# Autodesk Inventor assembly: ElevShortBackFrame
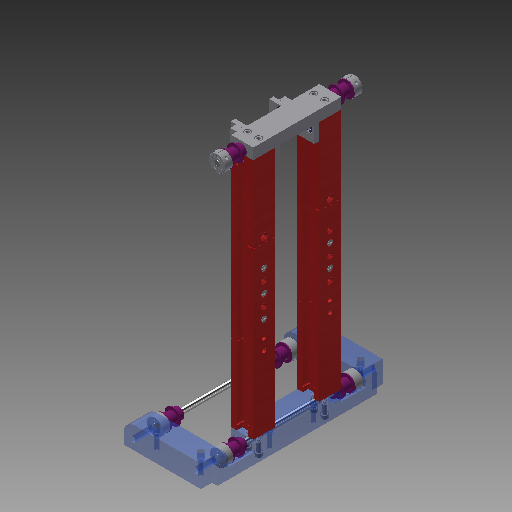
[picture p0: Inventor's stored thumbnail of the model, 512x512]
Saved by Autodesk Inventor 2019 (Build 230136000, 136)
## iProperties
Created: 2019-09-29
Part Number: ElevShortBackFrame
Document SubType Name: Weldment
Designer: james
Weld Material: Welded Aluminum-6061
Author: james
## Documents named in this file (9)
- F:\JimsDesign\Jims2020FTC\ElevShortBackFrame.iam
- F:\JimsDesign\Jims2020FTC\FullElevatorShart.iam
- F:\JimsDesign\Jims2020FTC\ElevBase.ipt
- F:\JimsDesign\Library\McMaster\SocketScrews\91251A201_BLACK-OXIDE ALLOY STEEL SOCKET HEAD SCREW.ipt
- F:\JimsDesign\Jims2020FTC\ElvatorEnd.iam
- F:\JimsDesign\Library\McMaster\Screws\91771A196_18-8 SS FLAT HEAD PHILLIPS MACHINE SCREW.ipt
- F:\JimsDesign\Jims2020FTC\SliderLeft.iam
- F:\JimsDesign\Jims2020FTC\SliderRight.iam
- F:\JimsDesign\Jims2020FTC\EvelShortBackBeam.iam
## Components (17 placed, 8 different names)
1. FullElevatorShart:1 [sub-assembly] — Mate:30, Mate:31
2. ElevBase:1 — Mate:11, Mate:12, Mate:13, Mate:14, Mate:15, Mate:16, Mate:17, Mate:18, Mate:19, Mate:20, Mate:26, Mate:33
3. FullElevatorShart:2 [sub-assembly] — Mate:11, Mate:12
4. EvelShortBackBeam:1 [sub-assembly] — Mate:22, Mate:25, Mate:26, Mate:28, Mate:29, Mate:38, Mate:39, Flush:1, Flush:2, Mate:44, Mate:45, Mate:46
5. EvelShortBackBeam:2 [sub-assembly] — Mate:34, Mate:35, Mate:36, Mate:37, Mate:40, Flush:3, Flush:4, Mate:41, Mate:42, Mate:43
6. 91251A201_BLACK-OXIDE ALLOY STEEL SOCKET HEAD SCREW:1 — Mate:16, Mate:17
7. 91251A201_BLACK-OXIDE ALLOY STEEL SOCKET HEAD SCREW:2 — Mate:15, Mate:19, Mate:22
8. 91251A201_BLACK-OXIDE ALLOY STEEL SOCKET HEAD SCREW:3 — Mate:14, Mate:20, Mate:25
9. 91251A201_BLACK-OXIDE ALLOY STEEL SOCKET HEAD SCREW:4 — Mate:13, Mate:18
10. ElvatorEnd:1 [sub-assembly] — Mate:28, Mate:29, Mate:30, Mate:31, Mate:32, Mate:34, Mate:35, Mate:36
11. FullElevatorShart:3 [sub-assembly] — Mate:32, Mate:33
12. 91771A196_18-8 SS FLAT HEAD PHILLIPS MACHINE SCREW:1 — Mate:39, Flush:2
13. 91771A196_18-8 SS FLAT HEAD PHILLIPS MACHINE SCREW:2 — Mate:38, Flush:1
14. 91771A196_18-8 SS FLAT HEAD PHILLIPS MACHINE SCREW:3 — Mate:40, Flush:4
15. 91771A196_18-8 SS FLAT HEAD PHILLIPS MACHINE SCREW:4 — Mate:37, Flush:3
16. SliderLeft:1 [sub-assembly] — Mate:41, Mate:42, Mate:43
17. SliderRight:1 [sub-assembly] — Mate:44, Mate:45, Mate:46
## Relationships (36: Mate 32, Flush 4)
- Mate:11: ElevBase:1 ↔ FullElevatorShart:2
- Mate:12: ElevBase:1 ↔ FullElevatorShart:2
- Mate:13: ElevBase:1 ↔ 91251A201_BLACK-OXIDE ALLOY STEEL SOCKET HEAD SCREW:4
- Mate:14: ElevBase:1 ↔ 91251A201_BLACK-OXIDE ALLOY STEEL SOCKET HEAD SCREW:3
- Mate:15: ElevBase:1 ↔ 91251A201_BLACK-OXIDE ALLOY STEEL SOCKET HEAD SCREW:2
- Mate:16: ElevBase:1 ↔ 91251A201_BLACK-OXIDE ALLOY STEEL SOCKET HEAD SCREW:1
- Mate:17: ElevBase:1 ↔ 91251A201_BLACK-OXIDE ALLOY STEEL SOCKET HEAD SCREW:1
- Mate:18: ElevBase:1 ↔ 91251A201_BLACK-OXIDE ALLOY STEEL SOCKET HEAD SCREW:4
- Mate:19: ElevBase:1 ↔ 91251A201_BLACK-OXIDE ALLOY STEEL SOCKET HEAD SCREW:2
- Mate:20: ElevBase:1 ↔ 91251A201_BLACK-OXIDE ALLOY STEEL SOCKET HEAD SCREW:3
- Mate:22: EvelShortBackBeam:1 ↔ 91251A201_BLACK-OXIDE ALLOY STEEL SOCKET HEAD SCREW:2
- Mate:25: EvelShortBackBeam:1 ↔ 91251A201_BLACK-OXIDE ALLOY STEEL SOCKET HEAD SCREW:3
- Mate:26: ElevBase:1 ↔ EvelShortBackBeam:1
- Mate:28: EvelShortBackBeam:1 ↔ ElvatorEnd:1
- Mate:29: EvelShortBackBeam:1 ↔ ElvatorEnd:1
- Mate:30: FullElevatorShart:1 ↔ ElvatorEnd:1
- Mate:31: FullElevatorShart:1 ↔ ElvatorEnd:1
- Mate:32: ElvatorEnd:1 ↔ FullElevatorShart:3
- Mate:33: ElevBase:1 ↔ FullElevatorShart:3
- Mate:34: EvelShortBackBeam:2 ↔ ElvatorEnd:1
- Mate:35: EvelShortBackBeam:2 ↔ ElvatorEnd:1
- Mate:36: EvelShortBackBeam:2 ↔ ElvatorEnd:1
- Mate:37: EvelShortBackBeam:2 ↔ 91771A196_18-8 SS FLAT HEAD PHILLIPS MACHINE SCREW:4
- Mate:38: EvelShortBackBeam:1 ↔ 91771A196_18-8 SS FLAT HEAD PHILLIPS MACHINE SCREW:2
- Mate:39: EvelShortBackBeam:1 ↔ 91771A196_18-8 SS FLAT HEAD PHILLIPS MACHINE SCREW:1
- Mate:40: EvelShortBackBeam:2 ↔ 91771A196_18-8 SS FLAT HEAD PHILLIPS MACHINE SCREW:3
- Flush:1: EvelShortBackBeam:1 ↔ 91771A196_18-8 SS FLAT HEAD PHILLIPS MACHINE SCREW:2
- Flush:2: EvelShortBackBeam:1 ↔ 91771A196_18-8 SS FLAT HEAD PHILLIPS MACHINE SCREW:1
- Flush:3: EvelShortBackBeam:2 ↔ 91771A196_18-8 SS FLAT HEAD PHILLIPS MACHINE SCREW:4
- Flush:4: EvelShortBackBeam:2 ↔ 91771A196_18-8 SS FLAT HEAD PHILLIPS MACHINE SCREW:3
- Mate:41: EvelShortBackBeam:2 ↔ SliderLeft:1
- Mate:42: EvelShortBackBeam:2 ↔ SliderLeft:1
- Mate:43: EvelShortBackBeam:2 ↔ SliderLeft:1
- Mate:44: EvelShortBackBeam:1 ↔ SliderRight:1
- Mate:45: EvelShortBackBeam:1 ↔ SliderRight:1
- Mate:46: EvelShortBackBeam:1 ↔ SliderRight:1
